# Autodesk Inventor assembly: LinearBearing
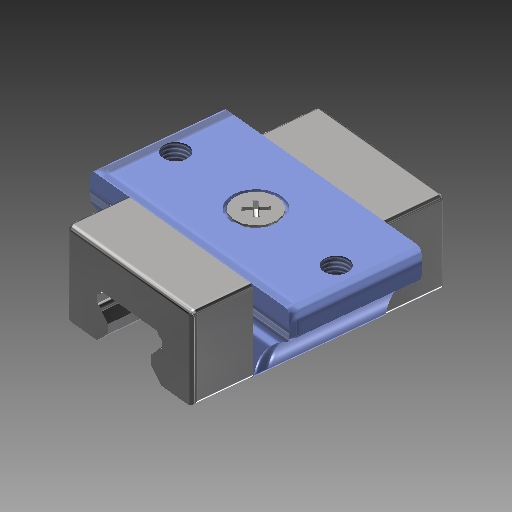
[picture p0: Inventor's stored thumbnail of the model, 512x512]
Saved by Autodesk Inventor 2018 (Build 220112000, 112)
## iProperties
Created: 2017-10-19
Part Number: LinearBearing
Document SubType Name: Assembly
Designer: Bryce Richards
Author: Bryce Richards
## Documents named in this file (4)
- E:\Mecanum\LinearBearing.iam
- E:\Mecanum\LinearSlide.ipt
- E:\Mecanum\LinearContact.ipt
- E:\Mecanum\Inventor\Content Center Files\R2018\en-US\AS 1427(04)\AS 1427 - M5 x 6(5) I.ipt
## Components (3 placed, 3 different names)
1. LinearSlide:1 — Mate:1, Mate:2, Mate:3, Mate:8
2. LinearContact:1 — Mate:1, Mate:2, Mate:3, Angle:2, Angle:3, Flush:1
3. AS 1427 H - Metric M5 x 6:1 — Angle:2, Angle:3, Mate:8, Flush:1
## Relationships (7: Mate 4, Angle 2, Flush 1)
- Mate:1: LinearSlide:1 ↔ LinearContact:1
- Mate:2: LinearSlide:1 ↔ LinearContact:1
- Mate:3: LinearSlide:1 ↔ LinearContact:1
- Angle:2 (0 deg): LinearContact:1 ↔ AS 1427 H - Metric M5 x 6:1
- Angle:3 (0 deg): LinearContact:1 ↔ AS 1427 H - Metric M5 x 6:1
- Mate:8: LinearSlide:1 ↔ AS 1427 H - Metric M5 x 6:1
- Flush:1: LinearContact:1 ↔ AS 1427 H - Metric M5 x 6:1
